# Autodesk Inventor assembly: Wheel Orientation
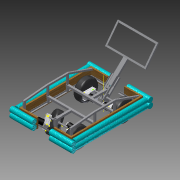
[picture p0: Inventor's stored thumbnail of the model, 180x180]
Saved by Autodesk Inventor 2015 (Build 190159000, 159)
## iProperties
Created: 2016-01-19
Part Number: Wheel Orientation
Document SubType Name: Assembly
Designer: sethbattis
Author: sethbattis
## Documents named in this file (11)
- \\area51\team3566\cad\FRC 2016\Space Claims.iam
- \\area51\team3566\cad\FRC 2016\Snow Blower Tire with Gear Box and Mini-CIM.iam
- \\area51\team3566\cad\FRC 2016\Side Bumper.ipt
- \\area51\team3566\cad\FRC 2016\Prow rev2.ipt
- \\area51\team3566\cad\FRC 2016\Catapult Base.ipt
- \\area51\team3566\cad\FRC 2016\Chassis.ipt
- \\area51\team3566\cad\FRC 2016\Top Axle.ipt
- \\area51\team3566\cad\FRC 2016\Snow Blower Tire with Gear Box and Mini-CIM_MIR1.iam
- \\area51\team3566\cad\FRC 2016\Snow Blower Tire with Gear Box and Mini-CIM_MIR2.iam
- \\area51\team3566\cad\FRC 2016\Top Axle_MIR.ipt
- \\area51\team3566\cad\FRC 2016\Snow Blower Tire with Gear Box and Mini-CIM_MIR1_MIR.iam
## Components (11 placed, 10 different names)
1. Chassis:1 — Mate:25, Mate:26, Mate:28, Mate:29, Mate:30, Mate:31, Mate:32, Mate:33, Mate:34, Mate:35, Mate:36, Mate:37, Mate:38, Mate:39
2. Prow rev2:1 — Mate:27, Mate:28
3. Catapult Base:1 — Mate:35, Mate:36
4. Top Axle:1 — Mate:25, Mate:26, Mate:27, Rotational:1, Rotational:2, Mate:39
5. Top Axle_MIR:1 — Rotational:3, Rotational:4, Mate:37, Mate:38
6. Snow Blower Tire with Gear Box and Mini-CIM_MIR2:1 [sub-assembly] — Rotational:3
7. Snow Blower Tire with Gear Box and Mini-CIM_MIR1_MIR:1 [sub-assembly] — Rotational:4
8. Snow Blower Tire with Gear Box and Mini-CIM:1 [sub-assembly] — Rotational:1
9. Snow Blower Tire with Gear Box and Mini-CIM_MIR1:1 [sub-assembly] — Rotational:2
10. Side Bumper:2 — Mate:32, Mate:33, Mate:34
11. Side Bumper:1 — Mate:29, Mate:30, Mate:31
## Relationships (19: Mate 15, RevoluteJoint 4)
- Mate:25: Chassis:1 ↔ Top Axle:1
- Mate:26: Chassis:1 ↔ Top Axle:1
- Mate:27: Prow rev2:1 ↔ Top Axle:1
- Mate:28: Chassis:1 ↔ Prow rev2:1
- Mate:29: Chassis:1 ↔ Side Bumper:1
- Mate:30: Chassis:1 ↔ Side Bumper:1
- Mate:31: Chassis:1 ↔ Side Bumper:1
- Mate:32: Chassis:1 ↔ Side Bumper:2
- Mate:33: Chassis:1 ↔ Side Bumper:2
- Mate:34: Chassis:1 ↔ Side Bumper:2
- Mate:35: Chassis:1 ↔ Catapult Base:1
- Mate:36: Chassis:1 ↔ Catapult Base:1
- Rotational:1 [RevoluteJoint]: Top Axle:1 ↔ Snow Blower Tire with Gear Box and Mini-CIM:1
- Rotational:2 [RevoluteJoint]: Top Axle:1 ↔ Snow Blower Tire with Gear Box and Mini-CIM_MIR1:1
- Rotational:3 [RevoluteJoint]: Top Axle_MIR:1 ↔ Snow Blower Tire with Gear Box and Mini-CIM_MIR2:1
- Rotational:4 [RevoluteJoint]: Top Axle_MIR:1 ↔ Snow Blower Tire with Gear Box and Mini-CIM_MIR1_MIR:1
- Mate:37: Chassis:1 ↔ Top Axle_MIR:1
- Mate:38: Chassis:1 ↔ Top Axle_MIR:1
- Mate:39: Chassis:1 ↔ Top Axle:1
